# Autodesk Inventor assembly: Z Motor Mount Assembly 1.0
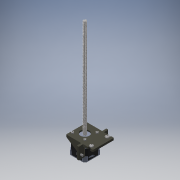
[picture p0: Inventor's stored thumbnail of the model, 180x180]
Saved by Autodesk Inventor 2016 (Build 200138000, 138)
## iProperties
Created: 2017-04-17
Part Number: Z Motor Mount Assembly 1.0
Document SubType Name: Assembly
Designer: Scott
Author: Scott
## Documents named in this file (5)
- E:\Scott Projects\3D Printing\CoreXY\Z Motor Mount Assembly 1.0.iam
- E:\Scott Projects\3D Printing\CoreXY\Z Motor Mount 1.0.ipt
- E:\Scott Projects\3D Printing\CoreXY\NEMA 17 T8x8 Assembly.iam
- C:\Users\Scott\Documents\Inventor\Content Center Files\R2016\en-US\ANSI B18.3.4M(1)\ANSI B18.3.4M - M5 x 0.8 x 10(2).ipt
- C:\Users\Scott\Documents\Inventor\Content Center Files\R2016\en-US\ANSI B18.3.1M(1)\ANSI B18.3.1M - M3x0.5 x 12(2).ipt
## Components (10 placed, 4 different names)
1. Z Motor Mount 1.0:1 — Insert:1, Angle:1, Insert:2, Insert:3, Insert:4, Insert:5, Insert:6, Insert:7, Insert:8, Insert:9
2. NEMA 17 T8x8 Assembly:1 [sub-assembly] — Insert:1, Angle:1
3. Broached Hexagon Socket Button Head Cap Screw - Metric M5 x 0.8 x 10:1 — Insert:5
4. Broached Hexagon Socket Button Head Cap Screw - Metric M5 x 0.8 x 10:2 — Insert:4
5. Broached Hexagon Socket Button Head Cap Screw - Metric M5 x 0.8 x 10:3 — Insert:3
6. Broached Hexagon Socket Button Head Cap Screw - Metric M5 x 0.8 x 10:4 — Insert:2
7. Broached Socket Head Cap Screw - Metric M3x0.5 x 12:1 — Insert:6
8. Broached Socket Head Cap Screw - Metric M3x0.5 x 12:2 — Insert:7
9. Broached Socket Head Cap Screw - Metric M3x0.5 x 12:3 — Insert:8
10. Broached Socket Head Cap Screw - Metric M3x0.5 x 12:4 — Insert:9
## Relationships (10: Insert 9, Angle 1)
- Insert:1: Z Motor Mount 1.0:1 ↔ NEMA 17 T8x8 Assembly:1
- Angle:1 (0 deg): Z Motor Mount 1.0:1 ↔ NEMA 17 T8x8 Assembly:1
- Insert:2: Z Motor Mount 1.0:1 ↔ Broached Hexagon Socket Button Head Cap Screw - Metric M5 x 0.8 x 10:4
- Insert:3: Z Motor Mount 1.0:1 ↔ Broached Hexagon Socket Button Head Cap Screw - Metric M5 x 0.8 x 10:3
- Insert:4: Z Motor Mount 1.0:1 ↔ Broached Hexagon Socket Button Head Cap Screw - Metric M5 x 0.8 x 10:2
- Insert:5: Z Motor Mount 1.0:1 ↔ Broached Hexagon Socket Button Head Cap Screw - Metric M5 x 0.8 x 10:1
- Insert:6: Z Motor Mount 1.0:1 ↔ Broached Socket Head Cap Screw - Metric M3x0.5 x 12:1
- Insert:7: Z Motor Mount 1.0:1 ↔ Broached Socket Head Cap Screw - Metric M3x0.5 x 12:2
- Insert:8: Z Motor Mount 1.0:1 ↔ Broached Socket Head Cap Screw - Metric M3x0.5 x 12:3
- Insert:9: Z Motor Mount 1.0:1 ↔ Broached Socket Head Cap Screw - Metric M3x0.5 x 12:4
